# Autodesk Inventor assembly: Lower Assembly 2
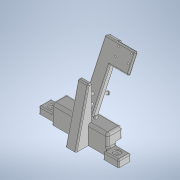
[picture p0: Inventor's stored thumbnail of the model, 180x180]
Saved by Autodesk Inventor 2020 (Build 240168000, 168)
## iProperties
Created: 2019-11-14
Part Number: Lower Assembly 2
Document SubType Name: Assembly
Designer: bzs3334
Author: bzs3334
## Documents named in this file (5)
- P:\GarbageGrader\3D Printed Parts\Lower Assembly 2.iam
- P:\GarbageGrader\3D Printed Parts\fakeM4Bolt.ipt
- P:\GarbageGrader\3D Printed Parts\fakeM4BoltLonger.ipt
- P:\GarbageGrader\3D Printed Parts\Lever V2.ipt
- P:\GarbageGrader\3D Printed Parts\Bottom Bracket + camera bottom thingy.ipt
## Components (4 placed, 4 different names)
1. fakeM4Bolt:1 — Mate:6, Mate:7
2. fakeM4BoltLonger:1 — Mate:8, Mate:9
3. Lever V2:1 — Mate:1, Mate:2, Mate:6, Mate:7, Mate:8
4. Bottom Bracket + camera bottom thingy:1 — Mate:1, Mate:2, Mate:3, Mate:4, Mate:5, Mate:9
## Relationships (9: Mate 9)
- Mate:1: Lever V2:1 ↔ Bottom Bracket + camera bottom thingy:1
- Mate:2: Lever V2:1 ↔ Bottom Bracket + camera bottom thingy:1
- Mate:3: Bottom Bracket + camera bottom thingy:1
- Mate:4: Bottom Bracket + camera bottom thingy:1
- Mate:5: Bottom Bracket + camera bottom thingy:1
- Mate:6: fakeM4Bolt:1 ↔ Lever V2:1
- Mate:7: fakeM4Bolt:1 ↔ Lever V2:1
- Mate:8: fakeM4BoltLonger:1 ↔ Lever V2:1
- Mate:9: fakeM4BoltLonger:1 ↔ Bottom Bracket + camera bottom thingy:1
